# Autodesk Inventor assembly: Main Piller And Support
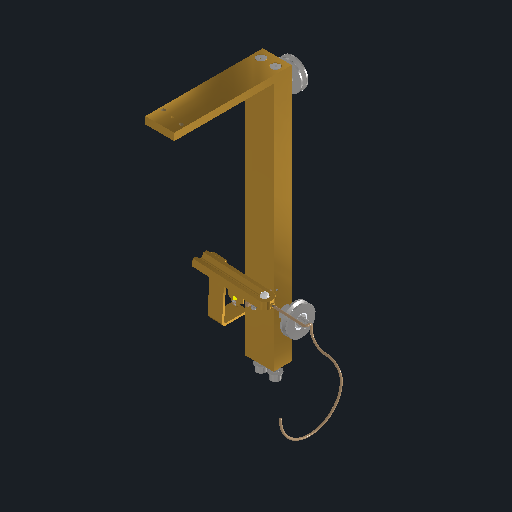
[picture p0: Inventor's stored thumbnail of the model, 512x512]
Saved by Autodesk Inventor 2027.1 (Build 311270010, 270A)
## iProperties
Created: 2025-09-16
Part Number: Main Piller And Support
Document SubType Name: Assembly
Designer: SD
Mass: 3689.38 g
Surface Area: 1072.9 cm^2
Volume: 461.49 cm^3
Density: 7.99449 g/cm^3
Project: Automatic Tea Steeping mechanism
BOM-Mass: 3.68938
BOM-Area: 0.107
Author: SD
Title: Main Piller And Support
## Documents named in this file (26)
- C:\Users\Gamer\Documents\Projects\Auto Tea Steeper\Public Version\Automatic Tea Steeper\CAD\Workspace\Main Piller And Support.iam
- C:\Users\Gamer\Documents\Projects\Auto Tea Steeper\Public Version\Automatic Tea Steeper\CAD\Workspace\Main Piller.ipt
- C:\Users\Gamer\Documents\Projects\Auto Tea Steeper\Public Version\Automatic Tea Steeper\CAD\Workspace\Support Beam.ipt
- C:\Users\Gamer\Documents\Projects\Auto Tea Steeper\Public Version\Automatic Tea Steeper\CAD\Workspace\Hardware\CSK Allen Key 6x25mm.ipt
- C:\Users\Gamer\Documents\Projects\Auto Tea Steeper\Public Version\Automatic Tea Steeper\CAD\Workspace\Hardware\Allen Key 8x25mm.ipt
- C:\Users\Gamer\Documents\Projects\Auto Tea Steeper\Public Version\Automatic Tea Steeper\CAD\Workspace\Pully Shaft.ipt
- C:\Users\Gamer\Documents\Projects\Auto Tea Steeper\Public Version\Automatic Tea Steeper\CAD\Workspace\Hardware\M10 Hex Nut.ipt
- C:\Users\Gamer\Documents\Projects\Auto Tea Steeper\Public Version\Automatic Tea Steeper\CAD\Workspace\Pully.ipt
- C:\Users\Gamer\Documents\Projects\Auto Tea Steeper\Public Version\Automatic Tea Steeper\CAD\Workspace\Hardware\19mm Circlips.ipt
- C:\Users\Gamer\Documents\Projects\Auto Tea Steeper\Public Version\Automatic Tea Steeper\CAD\Workspace\Hardware\61800 Bearing.ipt
- C:\Users\Gamer\Documents\Projects\Auto Tea Steeper\Public Version\Automatic Tea Steeper\CAD\Workspace\6mm Washer.ipt
- C:\Users\Gamer\Documents\Projects\Auto Tea Steeper\Public Version\Automatic Tea Steeper\CAD\Workspace\Hardware\CSK Allen Key 6x12mm.ipt
- C:\Users\Gamer\Documents\Projects\Auto Tea Steeper\Public Version\Automatic Tea Steeper\CAD\Workspace\Ball Track.ipt
- C:\Users\Gamer\Documents\Projects\Auto Tea Steeper\Public Version\Automatic Tea Steeper\CAD\Workspace\Ball Track Mounting Plate.ipt
- C:\Users\Gamer\Documents\Projects\Auto Tea Steeper\Public Version\Automatic Tea Steeper\CAD\Workspace\Ball Track Support.ipt
- C:\Users\Gamer\Documents\Projects\Auto Tea Steeper\Public Version\Automatic Tea Steeper\CAD\Workspace\Hardware\Brass M3 Hex Nut.ipt
- C:\Users\Gamer\Documents\Projects\Auto Tea Steeper\Public Version\Automatic Tea Steeper\CAD\Workspace\Hardware\3mm E Clip.ipt
- C:\Users\Gamer\Documents\Projects\Auto Tea Steeper\Public Version\Automatic Tea Steeper\CAD\Workspace\Platform.ipt
- C:\Users\Gamer\Documents\Projects\Auto Tea Steeper\Public Version\Automatic Tea Steeper\CAD\Workspace\Hardware\CSK Allen Key 3x8mm.ipt
- C:\Users\Gamer\Documents\Projects\Auto Tea Steeper\Public Version\Automatic Tea Steeper\CAD\Workspace\Hardware\Allen Key 3x5mm.ipt
- C:\Users\Gamer\Documents\Projects\Auto Tea Steeper\Public Version\Automatic Tea Steeper\CAD\Workspace\Ball.ipt
- C:\Users\Gamer\Documents\Projects\Auto Tea Steeper\Public Version\Automatic Tea Steeper\CAD\Workspace\Ball Track Rest Pin.ipt
- C:\Users\Gamer\Documents\Projects\Auto Tea Steeper\Public Version\Automatic Tea Steeper\CAD\Workspace\Hardware\8mm Washer.ipt
- C:\Users\Gamer\Documents\Projects\Auto Tea Steeper\Public Version\Automatic Tea Steeper\CAD\Workspace\Hardware\Grub Screw 3x3mm.ipt
- C:\Users\Gamer\Documents\Projects\Auto Tea Steeper\Public Version\Automatic Tea Steeper\CAD\Workspace\Hardware\Allen Key 3x10mm.ipt
- C:\Users\Gamer\Documents\Projects\Auto Tea Steeper\Public Version\Automatic Tea Steeper\CAD\Workspace\Tea Lifter Arm.ipt
## Components (38 placed, 25 different names)
1. Main Piller:1 — Flush:1, Mate:1, Mate:2, Mate:3, Mate:4, Mate:7, Mate:8, Mate:9, Mate:10, Mate:13, Mate:36, Mate:37, Mate:41, Mate:45, Mate:61, Flush:11, Mate:68, Mate:69, Angle:1
2. Support Beem:1 — Mate:2, Mate:3, Mate:4, Mate:5, Flush:2, Mate:6, Flush:3
3. CSK Allen Key 6x25mm:1 — Mate:5, Flush:2
4. CSK Allen Key 6x25mm:2 — Mate:6, Flush:3
5. Allen Key 8x25mm:1 — Mate:7, Flush:4, Mate:65, Mate:66
6. Allen Key 8x25mm:2 — Mate:8, Flush:4, Mate:9, Mate:64
7. Pully Shaft:1 — Mate:10, Mate:11, Mate:12, Mate:18, Mate:19, Mate:20, Mate:21
8. M10 Hex Nut:1 — Mate:11, Mate:12, Mate:13
9. Pully:1 — Mate:14, Mate:15, Mate:16, Mate:17, Mate:63
10. 19mm Circlips:1 — Mate:16, Mate:17, Mate:63
11. 61800 Bearing:1 — Mate:14, Mate:15, Mate:18, Mate:19
12. 6mm Washer:1 — Mate:20, Mate:21, Mate:22, Mate:23
13. Allen Key M6 x 12:1 — Mate:22, Mate:23
14. Pully Shaft:2 — Mate:25, Mate:36
15. M10 Hex Nut:2 — Mate:25, Mate:37
16. Pully:2 — Mate:67
17. 19mm Circlips:2 — Mate:67
18. 61800 Bearing:2
19. 6mm Washer:2
20. Allen Key M6 x 12:2
21. Ball Track:1 — Mate:38, Mate:39, Flush:5, Flush:8, Mate:57, Mate:58, Mate:62, Mate:71, Mate:72, Mate:73, Mate:75, Mate:76, Mate:77, Angle:2, Mate:79
22. Ball Track Mounting Plate:1 — Mate:38, Mate:39, Flush:5, Mate:42, Flush:6, Mate:55, Mate:56
23. Ball Track Support:1 — Mate:41, Mate:42, Mate:43, Mate:44, Flush:6, Mate:46, Mate:47, Mate:48, Mate:49
24. Brass M3 Hex Nut:1 — Mate:43, Mate:44, Mate:45
25. 3mm E Clip:1 — Mate:46, Mate:47
26. 3mm E Clip:2 — Mate:48, Mate:49
27. Platform:1 — Flush:8, Mate:71, Mate:72, Mate:73, Mate:74, Flush:14, Flush:15
28. CSK Allen Key 3x8mm:1 — Mate:74, Flush:14
29. CSK Allen Key 3x8mm:2 — Mate:75, Flush:15
30. ISO 4762 M3 x 5:1 — Mate:55, Mate:56
31. Ball:1 — Mate:57, Mate:58, Mate:62
32. Ball Track Rest Pin:1 — Mate:68, Mate:69, Angle:1, Mate:70, Flush:13
33. ISO 4026 M3 x 3:1 — Mate:61, Flush:11
34. ISO 7089 8:1 — Mate:65, Mate:66, Flush:12
35. ISO 7089 8:2 — Mate:64, Flush:12
36. ISO 4762 M3 x 10:1 — Mate:70, Flush:13
37. Tea Lifter Arm:1 — Mate:76, Mate:77, Angle:2, Mate:78
38. Brass M3 Hex Nut:2 — Mate:78, Mate:79
## Relationships (85: Mate 71, Flush 12, Angle 2)
- Flush:1: Main Piller:1
- Mate:1: Main Piller:1
- Mate:2: Main Piller:1 ↔ Support Beem:1
- Mate:3: Main Piller:1 ↔ Support Beem:1
- Mate:4: Main Piller:1 ↔ Support Beem:1
- Mate:5: Support Beem:1 ↔ CSK Allen Key 6x25mm:1
- Flush:2: Support Beem:1 ↔ CSK Allen Key 6x25mm:1
- Mate:6: Support Beem:1 ↔ CSK Allen Key 6x25mm:2
- Flush:3: Support Beem:1 ↔ CSK Allen Key 6x25mm:2
- Mate:7: Main Piller:1 ↔ Allen Key 8x25mm:1
- Mate:8: Main Piller:1 ↔ Allen Key 8x25mm:2
- Flush:4: Allen Key 8x25mm:1 ↔ Allen Key 8x25mm:2
- Mate:9 (11.5 mm): Main Piller:1 ↔ Allen Key 8x25mm:2
- Mate:10: Main Piller:1 ↔ Pully Shaft:1
- Mate:11: Pully Shaft:1 ↔ M10 Hex Nut:1
- Mate:12 (1 mm): Pully Shaft:1 ↔ M10 Hex Nut:1
- Mate:13: Main Piller:1 ↔ M10 Hex Nut:1
- Mate:14: Pully:1 ↔ 61800 Bearing:1
- Mate:15: Pully:1 ↔ 61800 Bearing:1
- Mate:16: Pully:1 ↔ 19mm Circlips:1
- Mate:17: Pully:1 ↔ 19mm Circlips:1
- Mate:18: Pully Shaft:1 ↔ 61800 Bearing:1
- Mate:19: Pully Shaft:1 ↔ 61800 Bearing:1
- Mate:20: Pully Shaft:1 ↔ 6mm Washer:1
- Mate:21: Pully Shaft:1 ↔ 6mm Washer:1
- Mate:22: 6mm Washer:1 ↔ Allen Key M6 x 12:1
- Mate:23: 6mm Washer:1 ↔ Allen Key M6 x 12:1
- [Mate]: Pully Shaft:2 ↔ M10 Hex Nut:2
- Mate:25 (1 mm): Pully Shaft:2 ↔ M10 Hex Nut:2
- [Mate]: Pully:2 ↔ 61800 Bearing:2
- [Mate]: Pully:2 ↔ 61800 Bearing:2
- [Mate]: Pully:2 ↔ 19mm Circlips:2
- [Mate]: Pully:2 ↔ 19mm Circlips:2
- [Mate]: Pully Shaft:2 ↔ 61800 Bearing:2
- [Mate]: Pully Shaft:2 ↔ 61800 Bearing:2
- [Mate]: Pully Shaft:2 ↔ 6mm Washer:2
- [Mate]: Pully Shaft:2 ↔ 6mm Washer:2
- [Mate]: 6mm Washer:2 ↔ Allen Key M6 x 12:2
- [Mate]: 6mm Washer:2 ↔ Allen Key M6 x 12:2
- Mate:36: Main Piller:1 ↔ Pully Shaft:2
- Mate:37: Main Piller:1 ↔ M10 Hex Nut:2
- Mate:38: Ball Track:1 ↔ Ball Track Mounting Plate:1
- Mate:39: Ball Track:1 ↔ Ball Track Mounting Plate:1
- Flush:5: Ball Track:1 ↔ Ball Track Mounting Plate:1
- Mate:41: Main Piller:1 ↔ Ball Track Support:1
- Mate:42: Ball Track Mounting Plate:1 ↔ Ball Track Support:1
- Mate:43: Ball Track Support:1 ↔ Brass M3 Hex Nut:1
- Mate:44 (-8 mm): Ball Track Support:1 ↔ Brass M3 Hex Nut:1
- Mate:45: Main Piller:1 ↔ Brass M3 Hex Nut:1
- Flush:6 (-0.5 mm): Ball Track Mounting Plate:1 ↔ Ball Track Support:1
- Mate:46: Ball Track Support:1 ↔ 3mm E Clip:1
- Mate:47: Ball Track Support:1 ↔ 3mm E Clip:1
- Mate:48: Ball Track Support:1 ↔ 3mm E Clip:2
- Mate:49: Ball Track Support:1 ↔ 3mm E Clip:2
- Flush:8 (5 mm): Ball Track:1 ↔ Platform:1
- Mate:55: Ball Track Mounting Plate:1 ↔ ISO 4762 M3 x 5:1
- Mate:56: Ball Track Mounting Plate:1 ↔ ISO 4762 M3 x 5:1
- Mate:57 (-1 mm): Ball Track:1 ↔ Ball:1
- Mate:58 (-10 mm): Ball Track:1 ↔ Ball:1
- Mate:61: Main Piller:1 ↔ ISO 4026 M3 x 3:1
- Flush:11 (0.5 mm): Main Piller:1 ↔ ISO 4026 M3 x 3:1
- Mate:62 (-10 mm): Ball Track:1 ↔ Ball:1
- Mate:63: Pully:1 ↔ 19mm Circlips:1
- Mate:64: Allen Key 8x25mm:2 ↔ ISO 7089 8:2
- Mate:65: Allen Key 8x25mm:1 ↔ ISO 7089 8:1
- Mate:66: Allen Key 8x25mm:1 ↔ ISO 7089 8:1
- Flush:12: ISO 7089 8:1 ↔ ISO 7089 8:2
- Mate:67: Pully:2 ↔ 19mm Circlips:2
- Mate:68: Main Piller:1 ↔ Ball Track Rest Pin:1
- Mate:69: Main Piller:1 ↔ Ball Track Rest Pin:1
- Angle:1 (0 deg): Main Piller:1 ↔ Ball Track Rest Pin:1
- Mate:70: Ball Track Rest Pin:1 ↔ ISO 4762 M3 x 10:1
- Flush:13 (7.5 mm): Ball Track Rest Pin:1 ↔ ISO 4762 M3 x 10:1
- Mate:71: Ball Track:1 ↔ Platform:1
- Mate:72: Ball Track:1 ↔ Platform:1
- Mate:73: Ball Track:1 ↔ Platform:1
- Mate:74: Platform:1 ↔ CSK Allen Key 3x8mm:1
- Flush:14: Platform:1 ↔ CSK Allen Key 3x8mm:1
- Mate:75: Ball Track:1 ↔ CSK Allen Key 3x8mm:2
- Flush:15: Platform:1 ↔ CSK Allen Key 3x8mm:2
- Mate:76: Ball Track:1 ↔ Tea Lifter Arm:1
- Mate:77 (-6 mm): Ball Track:1 ↔ Tea Lifter Arm:1
- Angle:2 (180 deg): Ball Track:1 ↔ Tea Lifter Arm:1
- Mate:78: Tea Lifter Arm:1 ↔ Brass M3 Hex Nut:2
- Mate:79: Ball Track:1 ↔ Brass M3 Hex Nut:2
## Named parameters: d28_d27 = 0 mm, d29_d17 = 0 mm, d30_d18 = 0 mm, d31_d19 = 0 mm, d32_d20 = 0 mm, d33_d21 = 0 mm, d34_d23 = 0 mm, d35_d24 = 0 mm, d36_d25 = 0 mm, d37_d26 = 0 mm, d38_d14 = 0 mm, d39_d15 = 1 mm
